# Autodesk Inventor assembly: SUB SYSTEM 1
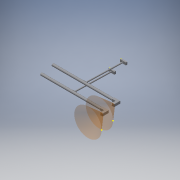
[picture p0: Inventor's stored thumbnail of the model, 180x180]
Saved by Autodesk Inventor 2018 (Build 220112000, 112)
## iProperties
Created: 2020-05-09
Part Number: SUB SYSTEM 1
Document SubType Name: Assembly
Designer: Darshan
Author: Darshan
## Documents named in this file (11)
- C:\Users\Darshan\Pictures\SUB SYSTEM 1.iam
- C:\Users\Darshan\Pictures\expofunl2_CPY.ipt
- C:\Users\Darshan\Pictures\expopipe.ipt
- C:\Users\Darshan\Pictures\elbow3_CPY.ipt
- C:\Users\Darshan\Pictures\Assembly5.iam
- C:\Users\Darshan\Pictures\base.ipt
- C:\Users\Darshan\Pictures\expofunl2_CPY_CPY.ipt
- C:\Users\Darshan\Pictures\expopipe_CPY2.ipt
- C:\Users\Darshan\Pictures\elbow3_CPY_CPY.ipt
- C:\Users\Darshan\Pictures\Assembly5_CPY.iam
- C:\Users\Darshan\Pictures\base_CPY.ipt
## Components (10 placed, 10 different names)
1. expofunl2_CPY:1 — Rigid:1
2. expopipe:1 — Rigid:2, Rigid:3
3. elbow3_CPY:1 — Rigid:1, Rigid:2
4. Assembly5:1 [sub-assembly] — Rigid:3, Rigid:4
5. base:1 — Rigid:4
6. expofunl2_CPY_CPY:1 — Rigid:6
7. expopipe_CPY2:1 — Rigid:5, Rigid:7
8. elbow3_CPY_CPY:1 — Rigid:5, Rigid:6
9. Assembly5_CPY:1 [sub-assembly] — Rigid:7, Rigid:8
10. base_CPY:1 — Rigid:8
## Relationships (8: WeldJoint 8)
- Rigid:1 [WeldJoint]: expofunl2_CPY:1 ↔ elbow3_CPY:1
- Rigid:2 [WeldJoint]: expopipe:1 ↔ elbow3_CPY:1
- Rigid:3 [WeldJoint]: expopipe:1 ↔ Assembly5:1
- Rigid:4 [WeldJoint]: Assembly5:1 ↔ base:1
- Rigid:5 [WeldJoint]: expopipe_CPY2:1 ↔ elbow3_CPY_CPY:1
- Rigid:6 [WeldJoint]: expofunl2_CPY_CPY:1 ↔ elbow3_CPY_CPY:1
- Rigid:7 [WeldJoint]: expopipe_CPY2:1 ↔ Assembly5_CPY:1
- Rigid:8 [WeldJoint]: Assembly5_CPY:1 ↔ base_CPY:1
